# Autodesk Inventor assembly: Assembly_Quenching
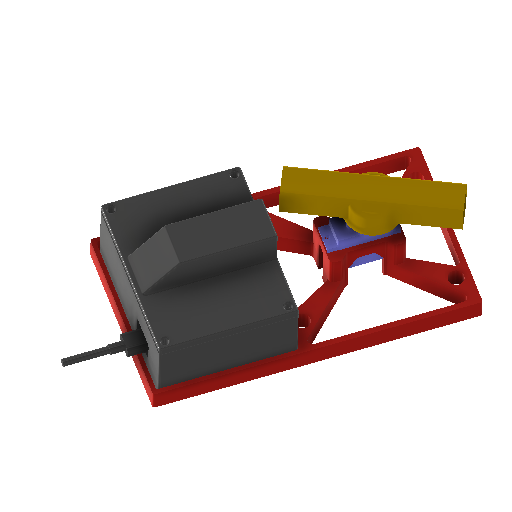
[picture p0: Inventor's stored thumbnail of the model, 512x512]
Saved by Autodesk Inventor 2026.1 (Build 301233020, 233B)
## iProperties
Created: 2026-01-21
Part Number: Assembly_Quenching
Document SubType Name: Assembly
Designer: samuel
Author: samuel
## Documents named in this file (3)
- E:\Fraunhofer\Design\Assembly_Quenching.iam
- E:\Fraunhofer\Design\Assembly_Box.iam
- E:\Fraunhofer\Design\Assembly_Servo.iam
## Components (2 placed, 2 different names)
1. Assembly_Box:1 [sub-assembly] — Mate:1, Mate:2, Flush:1
2. Assembly_Servo:1 [sub-assembly] — Mate:1, Mate:2, Flush:1
## Relationships (3: Mate 2, Flush 1)
- Mate:1: Assembly_Box:1 ↔ Assembly_Servo:1
- Mate:2: Assembly_Box:1 ↔ Assembly_Servo:1
- Flush:1: Assembly_Box:1 ↔ Assembly_Servo:1
